# Autodesk Inventor assembly: ЛЦМК000002.00.03.00.00.00 Наклонный вариант крепления
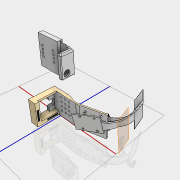
[picture p0: Inventor's stored thumbnail of the model, 180x180]
Saved by Autodesk Inventor 2021.2 (Build 252289000, 289)
## iProperties
Created: 2025-11-10
Part Number: ЛЦМК000002.00.03.00.00.00 Наклонный вариант крепления
Document SubType Name: Assembly
Designer: Захаров
Author: Захаров
## Documents named in this file (6)
- C:\Users\User\Documents\CaseARHead1\ЛЦМК000002.00.03.00.00.00 Наклонный вариант крепления.iam
- C:\Users\User\Documents\CaseARHead1\ЛЦМК000002.00.00.00.00.15.ipt
- C:\Users\User\Documents\CaseARHead1\ЛЦМК000002.00.00.00.00.18-01.ipt
- C:\Users\User\Documents\CaseARHead1\ЛЦМК000002.00.00.00.00.06-06.ipt
- C:\Users\User\Documents\CaseARHead1\ЛЦМК000002.00.00.00.00.13 OLED.ipt
- C:\Users\User\Documents\CaseARHead1\ЛЦМК000002.00.00.00.00.14 Фиксатор OLED.ipt
## Components (5 placed, 5 different names)
1. ЛЦМК000002.00.00.00.00.15:1 — Совмещение:1, Совмещение:2, Заподлицо:1
2. ЛЦМК000002.00.00.00.00.18-01:1 — Совмещение:1, Совмещение:2, Заподлицо:1
3. ЛЦМК000002.00.00.00.00.06-06:1 — Совмещение:3, Угол:1, Совмещение:4, Совмещение:5, Совмещение:6
4. ЛЦМК000002.00.00.00.00.13 OLED:1 — Совмещение:3, Угол:1
5. ЛЦМК000002.00.00.00.00.14 Фиксатор OLED:1 — Совмещение:4, Совмещение:5, Совмещение:6
## Relationships (8: Mate 6, Flush 1, Angle 1)
- Совмещение:1 [Mate]: ЛЦМК000002.00.00.00.00.15:1 ↔ ЛЦМК000002.00.00.00.00.18-01:1
- Совмещение:2 [Mate]: ЛЦМК000002.00.00.00.00.15:1 ↔ ЛЦМК000002.00.00.00.00.18-01:1
- Заподлицо:1 [Flush] (5 mm): ЛЦМК000002.00.00.00.00.15:1 ↔ ЛЦМК000002.00.00.00.00.18-01:1
- Совмещение:3 [Mate]: ЛЦМК000002.00.00.00.00.06-06:1 ↔ ЛЦМК000002.00.00.00.00.13 OLED:1
- Угол:1 [Angle] (-5.5 deg): ЛЦМК000002.00.00.00.00.06-06:1 ↔ ЛЦМК000002.00.00.00.00.13 OLED:1
- Совмещение:4 [Mate]: ЛЦМК000002.00.00.00.00.06-06:1 ↔ ЛЦМК000002.00.00.00.00.14 Фиксатор OLED:1
- Совмещение:5 [Mate]: ЛЦМК000002.00.00.00.00.06-06:1 ↔ ЛЦМК000002.00.00.00.00.14 Фиксатор OLED:1
- Совмещение:6 [Mate]: ЛЦМК000002.00.00.00.00.06-06:1 ↔ ЛЦМК000002.00.00.00.00.14 Фиксатор OLED:1
